# Autodesk Inventor assembly: ODSY-0004
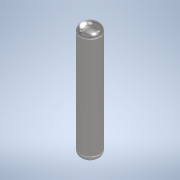
[picture p0: Inventor's stored thumbnail of the model, 180x180]
Saved by Autodesk Inventor 2021 (Build 250183000, 183)
## iProperties
Created: 2021-08-17
Part Number: ODSY-0004
Document SubType Name: Weldment
Designer: ALEX CLAY
Weld Material: Welded Aluminum-6061
Project: ODYSSEY
Description: OXIDIZER TANK
Mass: 156714 g
Surface Area: 43484.5 cm^2
Volume: 20278.4 cm^3
Density: 7.72811 g/cm^3
Author: ALEX CLAY
Title: OXIDIZER TANK
Revision Number: 00
## Documents named in this file (4)
- C:\Users\alexc\Embry-Riddle Aeronautical University\Kingsberry, Kyle A. - Odyssey\ATLAS V1\ODSY-0004 (TANK)\Weld Assembly.iam
- C:\Users\alexc\Embry-Riddle Aeronautical University\Kingsberry, Kyle A. - Odyssey\ATLAS V1\ODSY-0004 (TANK)\ODSY-0004-001.ipt
- C:\Users\alexc\Embry-Riddle Aeronautical University\Kingsberry, Kyle A. - Odyssey\ATLAS V1\ODSY-0004 (TANK)\ODSY-0004-002.ipt
- C:\Users\alexc\Embry-Riddle Aeronautical University\Kingsberry, Kyle A. - Odyssey\ATLAS V1\ODSY-0004 (TANK)\12555K74.ipt
## Components (5 placed, 3 different names)
1. ODSY-0004-001:1 — Flush:1, Mate:1, Mate:2, Mate:3, Mate:4, Mate:5
2. ODSY-0004-002:1 — Mate:2, Mate:3, Mate:22, Mate:23
3. ODSY-0004-002:2 — Mate:4, Mate:5, Mate:20, Mate:21
4. 12555K74:1 — Mate:22, Mate:23
5. 12555K74:2 — Mate:20, Mate:21
## Relationships (10: Mate 9, Flush 1)
- Flush:1: ODSY-0004-001:1
- Mate:1: ODSY-0004-001:1
- Mate:2: ODSY-0004-001:1 ↔ ODSY-0004-002:1
- Mate:3: ODSY-0004-001:1 ↔ ODSY-0004-002:1
- Mate:4: ODSY-0004-001:1 ↔ ODSY-0004-002:2
- Mate:5: ODSY-0004-001:1 ↔ ODSY-0004-002:2
- Mate:20: ODSY-0004-002:2 ↔ 12555K74:2
- Mate:21: ODSY-0004-002:2 ↔ 12555K74:2
- Mate:22: ODSY-0004-002:1 ↔ 12555K74:1
- Mate:23: ODSY-0004-002:1 ↔ 12555K74:1
